# Autodesk Inventor assembly: 3.25 Omni AS, No Insert_MIR
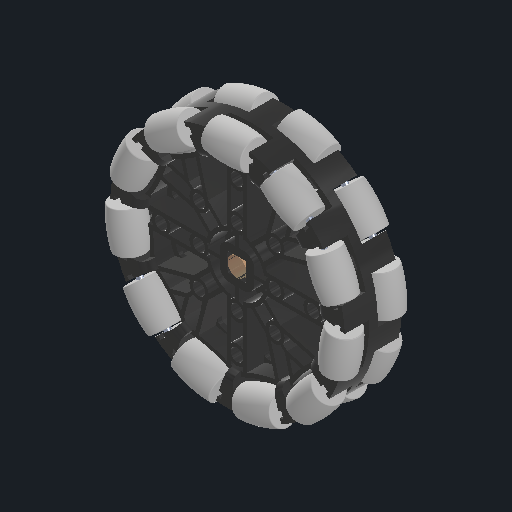
[picture p0: Inventor's stored thumbnail of the model, 512x512]
Saved by Autodesk Inventor 2024 (Build 280153000, 153)
## iProperties
Created: 2022-08-02
Part Number: 3.25 Omni AS, No Insert_MIR
Document SubType Name: Assembly
Designer: macbook
Author: ylu12
## Documents named in this file (2)
- \\Mac\Home\Desktop\code\1599V-VRC\Cad\Motion\Wheels\Omni Wheel\3.25 Omni AS, No Insert_MIR.iam
- \\Mac\Home\Desktop\code\1599V-VRC\Cad\Motion\Wheels\Reference Files\3.25 Omni Antistatic_MIR4.ipt
## Components (1 placed, 1 different names)
1. 3.25 Omni Antistatic_MIR4:1 — Mate:12, Mate:11, Flush:6
## Relationships (3: Mate 2, Flush 1)
- Mate:12: 3.25 Omni Antistatic_MIR4:1
- Mate:11: 3.25 Omni Antistatic_MIR4:1
- Flush:6: 3.25 Omni Antistatic_MIR4:1
